# Autodesk Inventor assembly: gripper_assembly
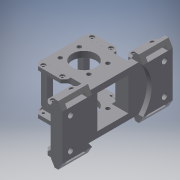
[picture p0: Inventor's stored thumbnail of the model, 180x180]
Saved by Autodesk Inventor 2016 (Build 200138000, 138)
## iProperties
Created: 2016-02-05
Part Number: gripper_assembly
Document SubType Name: Assembly
Designer: element
Mass: 43.7574 g
Surface Area: 218.602 cm^2
Volume: 43.7574 cm^3
Density: 1 g/cm^3
Author: element
## Documents named in this file (4)
- F:\technical_drawings\youbot\gripper\dynamixel_gripper\v2.0\inventor\motor_mount.iam
- F:\technical_drawings\youbot\gripper\dynamixel_gripper\v2.0\inventor\motor_base_plate.ipt
- F:\technical_drawings\youbot\gripper\dynamixel_gripper\v2.0\inventor\motor_brackets\brackets.iam
- F:\technical_drawings\youbot\gripper\dynamixel_gripper\v2.0\inventor\cable_tie_bracket.ipt
## Components (9 placed, 3 different names)
1. motor_base_plate:1 — Flush:24, Flush:25, Flush:26, Flush:27, Mate:31, Mate:32, Mate:33, Mate:34, Mate:35, Mate:36, Flush:28, Mate:37, Flush:31, Mate:42, Mate:43, Flush:32, Mate:45, Mate:46, Mate:47, Mate:48, Mate:49, Mate:50, Mate:51, Flush:33, Mate:52, Flush:34, Mate:53
2. brackets:1 [sub-assembly] — Flush:24, Mate:31, Mate:35
3. brackets:2 [sub-assembly] — Flush:25, Mate:32, Mate:36
4. brackets:3 [sub-assembly] — Flush:26, Mate:34, Flush:28
5. brackets:4 [sub-assembly] — Flush:27, Mate:33, Mate:37
6. cable_tie_bracket:1 — Mate:52, Flush:34, Mate:53
7. cable_tie_bracket:2 — Mate:50, Mate:51, Flush:33
8. cable_tie_bracket:3 — Mate:47, Mate:48, Mate:49
9. cable_tie_bracket:4 — Flush:32, Mate:45, Mate:46
## Relationships (27: Mate 18, Flush 9)
- Flush:24: motor_base_plate:1 ↔ brackets:1
- Flush:25: motor_base_plate:1 ↔ brackets:2
- Flush:26: motor_base_plate:1 ↔ brackets:3
- Flush:27: motor_base_plate:1 ↔ brackets:4
- Mate:31: motor_base_plate:1 ↔ brackets:1
- Mate:32: motor_base_plate:1 ↔ brackets:2
- Mate:33: motor_base_plate:1 ↔ brackets:4
- Mate:34: motor_base_plate:1 ↔ brackets:3
- Mate:35 (34 mm): motor_base_plate:1 ↔ brackets:1
- Mate:36 (-34 mm): motor_base_plate:1 ↔ brackets:2
- Flush:28 (-34 mm): motor_base_plate:1 ↔ brackets:3
- Mate:37 (34 mm): motor_base_plate:1 ↔ brackets:4
- Flush:31: motor_base_plate:1
- Mate:42: motor_base_plate:1
- Mate:43: motor_base_plate:1
- Flush:32: motor_base_plate:1 ↔ cable_tie_bracket:4
- Mate:45: motor_base_plate:1 ↔ cable_tie_bracket:4
- Mate:46: motor_base_plate:1 ↔ cable_tie_bracket:4
- Mate:47: motor_base_plate:1 ↔ cable_tie_bracket:3
- Mate:48: motor_base_plate:1 ↔ cable_tie_bracket:3
- Mate:49: motor_base_plate:1 ↔ cable_tie_bracket:3
- Mate:50: motor_base_plate:1 ↔ cable_tie_bracket:2
- Mate:51: motor_base_plate:1 ↔ cable_tie_bracket:2
- Flush:33: motor_base_plate:1 ↔ cable_tie_bracket:2
- Mate:52: motor_base_plate:1 ↔ cable_tie_bracket:1
- Flush:34: motor_base_plate:1 ↔ cable_tie_bracket:1
- Mate:53: motor_base_plate:1 ↔ cable_tie_bracket:1
